# Autodesk Inventor assembly: XcrRight
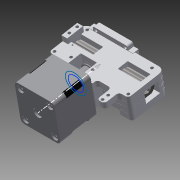
[picture p0: Inventor's stored thumbnail of the model, 180x180]
Saved by Autodesk Inventor 2013 (Build 170138000, 138)
## iProperties
Created: 2015-01-14
Part Number: XcrRight
Document SubType Name: Assembly
Designer: dzban
Author: dzban
## Documents named in this file (9)
- D:\PIRX\Artisan\OPENSOURCE\XCars\XcrRight.iam
- D:\PIRX\Artisan\OPENSOURCE\XCars\XcrRightXEndstopTrigger.ipt
- D:\PIRX\Artisan\OPENSOURCE\XCars\XcrRight_a.ipt
- D:\PIRX\Artisan\OPENSOURCE\XCars\XcrRight_b.ipt
- D:\PIRX\Artisan\OPENSOURCE\XCars\XcrRight_c.ipt
- D:\PIRX\Artisan\OPENSOURCE\XCars\XcrRightTop.ipt
- D:\PIRX\Artisan\OPENSOURCE\StockComponents\LM08UU.ipt
- D:\PIRX\Artisan\OPENSOURCE\StockComponents\NEMA17Stepper.ipt
- D:\PIRX\Artisan\OPENSOURCE\StockComponents\gt2_20_pulley.ipt
## Components (10 placed, 8 different names)
1. XcrRightXEndstopTrigger:1 — Insert:7, Insert:8
2. XcrRight_a:1 — Mate:1, Mate:2, Tangent:1, Tangent:2, Tangent:3, Tangent:4, Insert:1, Insert:2, Insert:7, Insert:8, Mate:3
3. XcrRight_b:1 — Insert:1, Insert:2, Insert:3, Insert:4, Mate:5
4. XcrRight_c:1 — Insert:5, Insert:6, Mate:4
5. XcrRightTop:1 — Mate:3, Mate:4, Mate:5, Insert:10, Insert:11
6. LM08UU:1 — Mate:1, Tangent:1, Tangent:2
7. LM08UU:2 — Mate:2, Tangent:3, Tangent:4
8. XcrRight_b:2 — Insert:3, Insert:4, Insert:5, Insert:6
9. NEMA17Stepper:1 — Insert:9, Insert:10, Insert:11
10. gt2_20_pulley:1 — Insert:9
## Relationships (20: Insert 11, Mate 5, Tangent 4)
- Mate:1: XcrRight_a:1 ↔ LM08UU:1
- Mate:2: XcrRight_a:1 ↔ LM08UU:2
- Tangent:1: XcrRight_a:1 ↔ LM08UU:1
- Tangent:2: XcrRight_a:1 ↔ LM08UU:1
- Tangent:3: XcrRight_a:1 ↔ LM08UU:2
- Tangent:4: XcrRight_a:1 ↔ LM08UU:2
- Insert:1: XcrRight_a:1 ↔ XcrRight_b:1
- Insert:2: XcrRight_a:1 ↔ XcrRight_b:1
- Insert:3: XcrRight_b:1 ↔ XcrRight_b:2
- Insert:4: XcrRight_b:1 ↔ XcrRight_b:2
- Insert:5: XcrRight_c:1 ↔ XcrRight_b:2
- Insert:6: XcrRight_c:1 ↔ XcrRight_b:2
- Insert:7: XcrRightXEndstopTrigger:1 ↔ XcrRight_a:1
- Insert:8: XcrRightXEndstopTrigger:1 ↔ XcrRight_a:1
- Mate:3: XcrRight_a:1 ↔ XcrRightTop:1
- Mate:4: XcrRight_c:1 ↔ XcrRightTop:1
- Mate:5: XcrRight_b:1 ↔ XcrRightTop:1
- Insert:9: NEMA17Stepper:1 ↔ gt2_20_pulley:1
- Insert:10 (42 mm): XcrRightTop:1 ↔ NEMA17Stepper:1
- Insert:11 (42 mm): XcrRightTop:1 ↔ NEMA17Stepper:1
